# Autodesk Inventor assembly: Zespół1
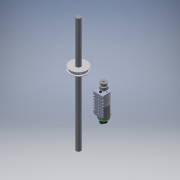
[picture p0: Inventor's stored thumbnail of the model, 180x180]
Saved by Autodesk Inventor 2019.4 (Build 234330000, 330)
## iProperties
Created: 2020-05-17
Part Number: Zespół1
Material: Ogólny
Document SubType Name: Assembly
Designer: barto
Author: barto
## Documents named in this file (7)
- F:\MUM\Zespół1.iam
- C:\Users\barto\Downloads\pololu-25d-mm-metal-gearmotor-bracket.ipt
- F:\MUM\25d-metal-gearmotor-378-499-encoder.ipt
- F:\MUM\kolooooo.ipt
- C:\Users\barto\OneDrive\Dokumenty\Inventor\Content Center Files\R2019\pl-PL\ISO 7045  H\ISO 7045 - M3 x 6 - 4.8 - H - ISO.ipt
- F:\MUM\GT2 pulley 60 teeth width 11mm 8mm bore.ipt
- F:\MUM\pret.ipt
## Components (7 placed, 6 different names)
1. pololu-25d-mm-metal-gearmotor-bracket:1 — Zestawiające:1, Zestawiające:2, Zestawiające:3, Zestawiające:6, Zestawiające:7, Zestawiające:8, Zestawiające:9
2. 25d-metal-gearmotor-378-499-encoder:1 — Zestawiające:1, Zestawiające:2, Zestawiające:3, Zestawiające:4, Zestawiające:5
3. kolooooo:1 — Zestawiające:4, Zestawiające:9, Równoległe:1
4. ISO 7045 H M3 x 6 - 4.8 - H:1 — Zestawiające:5, Zestawiające:6
5. ISO 7045 H M3 x 6 - 4.8 - H:2 — Zestawiające:7, Zestawiające:8
6. GT2 pulley 60 teeth width 11mm 8mm bore:1 — Równoległe:1, Zestawiające:10
7. pret:1 — Zestawiające:10
## Relationships (11: Mate 10, Flush 1)
- Zestawiające:1 [Mate]: pololu-25d-mm-metal-gearmotor-bracket:1 ↔ 25d-metal-gearmotor-378-499-encoder:1
- Zestawiające:2 [Mate]: pololu-25d-mm-metal-gearmotor-bracket:1 ↔ 25d-metal-gearmotor-378-499-encoder:1
- Zestawiające:3 [Mate]: pololu-25d-mm-metal-gearmotor-bracket:1 ↔ 25d-metal-gearmotor-378-499-encoder:1
- Zestawiające:4 [Mate]: 25d-metal-gearmotor-378-499-encoder:1 ↔ kolooooo:1
- Zestawiające:5 [Mate]: 25d-metal-gearmotor-378-499-encoder:1 ↔ ISO 7045 H M3 x 6 - 4.8 - H:1
- Zestawiające:6 [Mate]: pololu-25d-mm-metal-gearmotor-bracket:1 ↔ ISO 7045 H M3 x 6 - 4.8 - H:1
- Zestawiające:7 [Mate]: pololu-25d-mm-metal-gearmotor-bracket:1 ↔ ISO 7045 H M3 x 6 - 4.8 - H:2
- Zestawiające:8 [Mate]: pololu-25d-mm-metal-gearmotor-bracket:1 ↔ ISO 7045 H M3 x 6 - 4.8 - H:2
- Zestawiające:9 [Mate] (3.5 mm): pololu-25d-mm-metal-gearmotor-bracket:1 ↔ kolooooo:1
- Równoległe:1 [Flush]: kolooooo:1 ↔ GT2 pulley 60 teeth width 11mm 8mm bore:1
- Zestawiające:10 [Mate]: GT2 pulley 60 teeth width 11mm 8mm bore:1 ↔ pret:1
